# Autodesk Inventor assembly: DIFF_HOUSING_FINAL_ASM
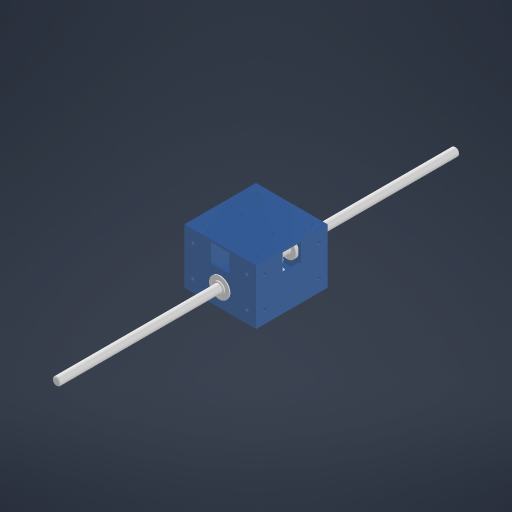
[picture p0: Inventor's stored thumbnail of the model, 512x512]
Saved by Autodesk Inventor 2024 (Build 280153000, 153)
## iProperties
Created: 2023-11-30
Part Number: DIFF_HOUSING_FINAL_ASM
Document SubType Name: Assembly
Designer: bugme
Author: bugme
## Documents named in this file (8)
- C:\Users\bugme\OneDrive - The Pennsylvania State University\Desktop\BRCRP\DIFF_HOUSING_FINAL_ASM.iam
- C:\Users\bugme\OneDrive - The Pennsylvania State University\Desktop\BRCRP\DIFF_HOUSING_WIP.ipt
- C:\Users\bugme\OneDrive - The Pennsylvania State University\Desktop\BRCRP\CH-1-01-20x20 Channel.ipt
- C:\Users\bugme\OneDrive - The Pennsylvania State University\Desktop\BRCRP\DIFF_HOUSING_TOP.ipt
- C:\Users\bugme\OneDrive - The Pennsylvania State University\Desktop\BRCRP\CH-1-01-20x20 Channel\CH-1-01-20x20 Channel-3.13.ipt
- C:\Users\bugme\OneDrive - The Pennsylvania State University\Desktop\BRCRP\6384K361_Ball Bearing\6384K361_Ball Bearing.ipt
- C:\Users\bugme\OneDrive - The Pennsylvania State University\Desktop\BRCRP\1886K21_Rotary Shaft (1)\1886K21_Rotary Shaft (1).ipt
- C:\Users\bugme\OneDrive - The Pennsylvania State University\Desktop\BRCRP\6529K15_Metal Miter Gear (2)\6529K15_Metal Miter Gear (2).ipt
## Components (14 placed, 6 different names)
1. DIFF_HOUSING_WIP:1 — Mate:1, Mate:2, Flush:1, Mate:3, Mate:4, Flush:2, Mate:5, Mate:6, Flush:3, Mate:7, Mate:8, Flush:4, Flush:5, Flush:6, Flush:7, Flush:8, Mate:11, Mate:12, Mate:13, Mate:14, Flush:9, Flush:10, Mate:19
2. CH-1-01-20x20 Channel-3.13:1 — Mate:1, Mate:2, Flush:1, Mate:10
3. CH-1-01-20x20 Channel-3.13:2 — Mate:3, Mate:4, Flush:2, Mate:9
4. CH-1-01-20x20 Channel-3.13:3 — Mate:5, Mate:6, Flush:3
5. CH-1-01-20x20 Channel-3.13:4 — Mate:7, Mate:8, Flush:4
6. DIFF_HOUSING_TOP:1 — Mate:9, Flush:5, Flush:6
7. DIFF_HOUSING_TOP:2 — Mate:10, Flush:7, Flush:8
8. 6384K361_Ball Bearing:1 — Mate:11, Mate:12, Mate:15
9. 6384K361_Ball Bearing:2 — Mate:13, Mate:14, Mate:16
10. 1886K21_Rotary Shaft (1):1 — Mate:15, Flush:9, Mate:17
11. 1886K21_Rotary Shaft (1):2 — Mate:16, Flush:10, Mate:18
12. 6529K15_Metal Miter Gear (2):1 — Mate:17
13. 6529K15_Metal Miter Gear (2):2 — Mate:18, Mate:20
14. 6529K15_Metal Miter Gear (2):3 — Mate:19, Mate:20
## Relationships (30: Mate 20, Flush 10)
- Mate:1: DIFF_HOUSING_WIP:1 ↔ CH-1-01-20x20 Channel-3.13:1
- Mate:2: DIFF_HOUSING_WIP:1 ↔ CH-1-01-20x20 Channel-3.13:1
- Flush:1: DIFF_HOUSING_WIP:1 ↔ CH-1-01-20x20 Channel-3.13:1
- Mate:3: DIFF_HOUSING_WIP:1 ↔ CH-1-01-20x20 Channel-3.13:2
- Mate:4: DIFF_HOUSING_WIP:1 ↔ CH-1-01-20x20 Channel-3.13:2
- Flush:2: DIFF_HOUSING_WIP:1 ↔ CH-1-01-20x20 Channel-3.13:2
- Mate:5: DIFF_HOUSING_WIP:1 ↔ CH-1-01-20x20 Channel-3.13:3
- Mate:6: DIFF_HOUSING_WIP:1 ↔ CH-1-01-20x20 Channel-3.13:3
- Flush:3: DIFF_HOUSING_WIP:1 ↔ CH-1-01-20x20 Channel-3.13:3
- Mate:7: DIFF_HOUSING_WIP:1 ↔ CH-1-01-20x20 Channel-3.13:4
- Mate:8: DIFF_HOUSING_WIP:1 ↔ CH-1-01-20x20 Channel-3.13:4
- Flush:4: DIFF_HOUSING_WIP:1 ↔ CH-1-01-20x20 Channel-3.13:4
- Mate:9: CH-1-01-20x20 Channel-3.13:2 ↔ DIFF_HOUSING_TOP:1
- Flush:5: DIFF_HOUSING_WIP:1 ↔ DIFF_HOUSING_TOP:1
- Flush:6: DIFF_HOUSING_WIP:1 ↔ DIFF_HOUSING_TOP:1
- Mate:10: CH-1-01-20x20 Channel-3.13:1 ↔ DIFF_HOUSING_TOP:2
- Flush:7: DIFF_HOUSING_WIP:1 ↔ DIFF_HOUSING_TOP:2
- Flush:8: DIFF_HOUSING_WIP:1 ↔ DIFF_HOUSING_TOP:2
- Mate:11: DIFF_HOUSING_WIP:1 ↔ 6384K361_Ball Bearing:1
- Mate:12: DIFF_HOUSING_WIP:1 ↔ 6384K361_Ball Bearing:1
- Mate:13: DIFF_HOUSING_WIP:1 ↔ 6384K361_Ball Bearing:2
- Mate:14: DIFF_HOUSING_WIP:1 ↔ 6384K361_Ball Bearing:2
- Mate:15: 6384K361_Ball Bearing:1 ↔ 1886K21_Rotary Shaft (1):1
- Flush:9 (-45.72 mm): DIFF_HOUSING_WIP:1 ↔ 1886K21_Rotary Shaft (1):1
- Mate:16: 6384K361_Ball Bearing:2 ↔ 1886K21_Rotary Shaft (1):2
- Flush:10 (-45.72 mm): DIFF_HOUSING_WIP:1 ↔ 1886K21_Rotary Shaft (1):2
- Mate:17: 1886K21_Rotary Shaft (1):1 ↔ 6529K15_Metal Miter Gear (2):1
- Mate:18: 1886K21_Rotary Shaft (1):2 ↔ 6529K15_Metal Miter Gear (2):2
- Mate:19: DIFF_HOUSING_WIP:1 ↔ 6529K15_Metal Miter Gear (2):3
- Mate:20: 6529K15_Metal Miter Gear (2):2 ↔ 6529K15_Metal Miter Gear (2):3
